# Autodesk Inventor assembly: Manual_robot_design_draft
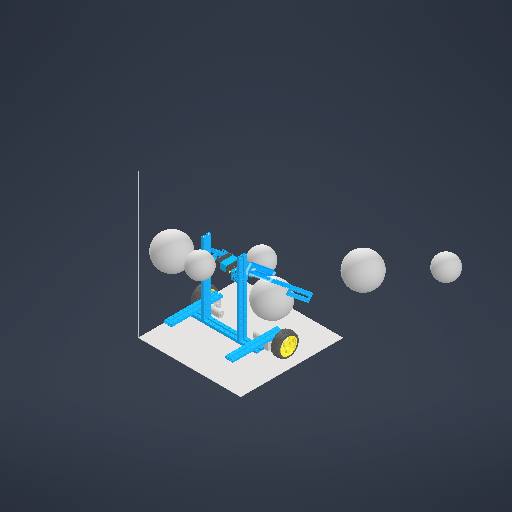
[picture p0: Inventor's stored thumbnail of the model, 512x512]
Saved by Autodesk Inventor 2026.1 (Build 301233020, 233B)
## iProperties
Created: 2025-10-16
Part Number: Manual_robot_design_draft
Document SubType Name: Assembly
Designer: Asus
Author: Asus
## Documents named in this file (16)
- D:\KMITL\Computer_Programming\ComPro_Project\Robot_design_CAD_files\Full_Manual_Robot_Assembly_V1_23.10.25.iam
- D:\KMITL\Computer_Programming\ComPro_Project\Material_Parts_CAD_files\Metal_parts\Beam0824-224.ipt
- D:\KMITL\Computer_Programming\ComPro_Project\Field_materials_CAD_files\Manual_Robot_Size_Base.ipt
- D:\KMITL\Computer_Programming\ComPro_Project\Field_materials_CAD_files\Objective_70mm_Ball_Manual.ipt
- D:\KMITL\Computer_Programming\ComPro_Project\Field_materials_CAD_files\Objective_100mm_Ball_Manual.ipt
- D:\KMITL\Computer_Programming\ComPro_Project\Material_Parts_CAD_files\Metal_parts\Beam9x8x1-136.ipt
- D:\KMITL\Computer_Programming\ComPro_Project\Material_Parts_CAD_files\Metal_parts\Beam0824-160.ipt
- D:\KMITL\Computer_Programming\ComPro_Project\Material_Parts_CAD_files\MakeX_parts\Encoder Motor.ipt
- D:\KMITL\Computer_Programming\ComPro_Project\Material_Parts_CAD_files\Arudino_parts\Wheel D65x25.ipt
- D:\KMITL\Computer_Programming\ComPro_Project\Material_Parts_CAD_files\Metal_parts\Plate0324-088 V1.0.ipt
- D:\KMITL\Computer_Programming\ComPro_Project\Material_Parts_CAD_files\Metal_parts\U-Shape_Bracket.ipt
- D:\KMITL\Computer_Programming\ComPro_Project\Material_Parts_CAD_files\Electronic_parts\MEDS15 - Servo Motor.ipt
- D:\KMITL\Computer_Programming\ComPro_Project\Material_Parts_CAD_files\Metal_parts\Bracket 3x3.ipt
- D:\KMITL\Computer_Programming\ComPro_Project\Material_Parts_CAD_files\Metal_parts\Plate0324-072 V1.0.ipt
- D:\KMITL\Computer_Programming\ComPro_Project\Material_Parts_CAD_files\Metal_parts\Beam0824-032.ipt
- D:\KMITL\Computer_Programming\ComPro_Project\Field_materials_CAD_files\Manual_Robot_Height_Limit.ipt
## Components (31 placed, 15 different names)
1. Beam0824-224:3 — Rigid:4, Rigid:5, Rigid:8, Rigid:10
2. Beam0824-224:4 — Rigid:8, Rigid:11
3. Manual_Robot_Size_Base:1 — Flush:3, Tangent:3, Tangent:4, Mate:1, Rigid:22
4. Objective_70mm_Ball_Manual:1 — Tangent:1
5. Objective_100mm_Ball_Manual:1 — Tangent:2
6. Beam9x8x1-136:1 — Rigid:3, Rigid:17
7. Beam9x8x1-136:2 — Rigid:3, Rigid:9
8. Objective_100mm_Ball_Manual:2 — Tangent:3
9. Objective_70mm_Ball_Manual:2 — Tangent:4
10. Objective_100mm_Ball_Manual:3
11. Objective_70mm_Ball_Manual:3
12. Beam0824-160:1 — Rigid:4, Rigid:6
13. Beam0824-160:2 — Rigid:5, Rigid:7
14. Encoder Motor:1 — Rigid:7, Rotational:2
15. Encoder Motor:2 — Rigid:6, Rotational:1, Mate:1
16. Wheel D65x25:1 — Rotational:2
17. Wheel D65x25:2 — Rotational:1
18. Plate0324-088 V1.0:1 — Rigid:9
19. U-Shape_Bracket:1 — Rigid:11, Rigid:13
20. U-Shape_Bracket:2 — Rigid:12
21. MEDS15 - Servo Motor:1 — Rigid:13, Rotational:3
22. Beam0824-224:5 — Rigid:10, Rigid:12
23. Bracket 3x3:1 — Rigid:14, Rigid:18
24. Bracket 3x3:2 — Rigid:15, Rotational:3, Rigid:16
25. Plate0324-072 V1.0:1 — Rigid:14, Rigid:15
26. Beam0824-032:1 — Rigid:16, Rigid:17
27. Beam0824-032:2 — Rigid:18, Rigid:21
28. Beam9x8x1-136:3 — Rigid:19, Rigid:21
29. Beam9x8x1-136:4 — Rigid:19, Rigid:20
30. Plate0324-088 V1.0:2 — Rigid:20
31. Manual_Robot_Height_Limit:1 — Rigid:22
## Relationships (31: WeldJoint 20, Tangent 4, Flush 3, RevoluteJoint 3, Mate 1)
- Flush:1 (-320 mm)
- Flush:2 (-320 mm)
- Flush:3 (136 mm): Manual_Robot_Size_Base:1
- Tangent:1: Objective_70mm_Ball_Manual:1
- Tangent:2: Objective_100mm_Ball_Manual:1
- Tangent:3: Manual_Robot_Size_Base:1 ↔ Objective_100mm_Ball_Manual:2
- Tangent:4: Manual_Robot_Size_Base:1 ↔ Objective_70mm_Ball_Manual:2
- Rigid:3 [WeldJoint]: Beam9x8x1-136:1 ↔ Beam9x8x1-136:2
- Rigid:4 [WeldJoint]: Beam0824-224:3 ↔ Beam0824-160:1
- Rigid:5 [WeldJoint]: Beam0824-224:3 ↔ Beam0824-160:2
- Rigid:6 [WeldJoint]: Beam0824-160:1 ↔ Encoder Motor:2
- Rigid:7 [WeldJoint]: Beam0824-160:2 ↔ Encoder Motor:1
- Rotational:1 [RevoluteJoint]: Encoder Motor:2 ↔ Wheel D65x25:2
- Rotational:2 [RevoluteJoint]: Encoder Motor:1 ↔ Wheel D65x25:1
- Mate:1 (20.5 mm): Manual_Robot_Size_Base:1 ↔ Encoder Motor:2
- Rigid:8 [WeldJoint]: Beam0824-224:3 ↔ Beam0824-224:4
- Rigid:9 [WeldJoint]: Beam9x8x1-136:2 ↔ Plate0324-088 V1.0:1
- Rigid:10 [WeldJoint]: Beam0824-224:3 ↔ Beam0824-224:5
- Rigid:11 [WeldJoint]: Beam0824-224:4 ↔ U-Shape_Bracket:1
- Rigid:12 [WeldJoint]: U-Shape_Bracket:2 ↔ Beam0824-224:5
- Rigid:13 [WeldJoint] (-7.9 mm): U-Shape_Bracket:1 ↔ MEDS15 - Servo Motor:1
- Rigid:14 [WeldJoint]: Bracket 3x3:1 ↔ Plate0324-072 V1.0:1
- Rigid:15 [WeldJoint]: Bracket 3x3:2 ↔ Plate0324-072 V1.0:1
- Rotational:3 [RevoluteJoint]: MEDS15 - Servo Motor:1 ↔ Bracket 3x3:2
- Rigid:16 [WeldJoint]: Bracket 3x3:2 ↔ Beam0824-032:1
- Rigid:17 [WeldJoint]: Beam9x8x1-136:1 ↔ Beam0824-032:1
- Rigid:18 [WeldJoint]: Bracket 3x3:1 ↔ Beam0824-032:2
- Rigid:19 [WeldJoint]: Beam9x8x1-136:3 ↔ Beam9x8x1-136:4
- Rigid:20 [WeldJoint]: Beam9x8x1-136:4 ↔ Plate0324-088 V1.0:2
- Rigid:21 [WeldJoint]: Beam0824-032:2 ↔ Beam9x8x1-136:3
- Rigid:22 [WeldJoint]: Manual_Robot_Size_Base:1 ↔ Manual_Robot_Height_Limit:1
## Named parameters: d54_d24 = 0 mm, d55_d37 = 0 mm
